# Autodesk Inventor assembly: 275-1272-STEP
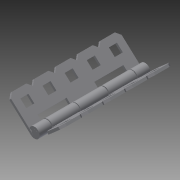
[picture p0: Inventor's stored thumbnail of the model, 180x180]
Saved by Autodesk Inventor 2014 SP1 (Build 180222100, 222)
## iProperties
Created: 2014-02-27
Part Number: 275-1272-STEP
Document SubType Name: Assembly
Designer: Ryan
Title: VEX-HINGE-ASM.STEP
Description: STEP AP203
Creation Date: 2011-01-25
Sending System: SolidWorks 2010
Preprocessor: SwSTEP 2.0
Author: Ryan
## Documents named in this file (4)
- C:\Users\Ryan\Desktop\sw\lib\Aperture VEX CAD Library\Metal\vex hinge\hinge.iam
- C:\Users\Ryan\Desktop\sw\lib\Aperture VEX CAD Library\Metal\vex hinge\parts\VEX-HINGE-PIN.ipt
- C:\Users\Ryan\Desktop\sw\lib\Aperture VEX CAD Library\Metal\vex hinge\parts\VEX-HINGE-1 RevA.ipt
- C:\Users\Ryan\Desktop\sw\lib\Aperture VEX CAD Library\Metal\vex hinge\parts\VEX-HINGE-2 RevA.ipt
## Components (3 placed, 3 different names)
1. VEX-HINGE-PIN_1 — Mate:2, Flush:2
2. VEX-HINGE-1 RevA_2 — Mate:1, Mate:2, Flush:1, Flush:2
3. VEX-HINGE-2 RevA_3 — Mate:1, Flush:1
## Relationships (4: Mate 2, Flush 2)
- Mate:1: VEX-HINGE-1 RevA_2 ↔ VEX-HINGE-2 RevA_3
- Mate:2: VEX-HINGE-PIN_1 ↔ VEX-HINGE-1 RevA_2
- Flush:1: VEX-HINGE-1 RevA_2 ↔ VEX-HINGE-2 RevA_3
- Flush:2: VEX-HINGE-PIN_1 ↔ VEX-HINGE-1 RevA_2
